# Autodesk Inventor assembly: Traction_Section
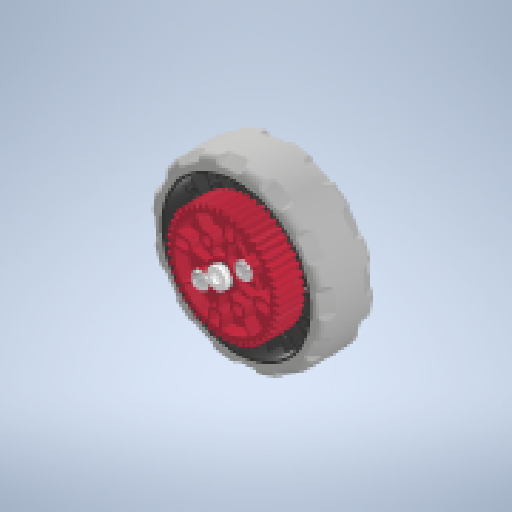
[picture p0: Inventor's stored thumbnail of the model, 512x512]
Saved by Autodesk Inventor 2025.2 (Build 292293000, 293)
## iProperties
Created: 2024-12-08
Part Number: Traction_Section
Document SubType Name: Assembly
Designer: Aditya Koduri
Author: Aditya Koduri
## Documents named in this file (13)
- C:\Users\joshi\Desktop\3388K CAD\Traction_Section.iam
- C:\Users\joshi\Desktop\3388K CAD\VEX Main\Structure\Hardware\Screw Steel - Hex\SScrew Hex Smooth 1.250.ipt
- C:\Users\joshi\Desktop\3388K CAD\VEX Main\Motion\Gears\HS Gear\HS 48T Gear, No Insert.iam
- C:\Users\joshi\Desktop\3388K CAD\VEX Main\Structure\Hardware\Nut Thin Nylock.ipt
- C:\Users\joshi\Desktop\3388K CAD\VEX Main\Motion\Wheels\Traction Wheel\3.25 Traction AS, No Insert.iam
- C:\Users\joshi\Desktop\3388K CAD\VEX Main\Motion\Insert Circle.ipt
- C:\Users\joshi\Desktop\3388K CAD\VEX Main\Motion\Spacers\Washer Teflon\TWasher .375 OD x .03125.ipt
- C:\Users\joshi\Desktop\3388K CAD\VEX Main\Motion\Spacers\Spacer Nylon .313 OD\NSpacer .313 OD x .250.ipt
- C:\Users\mzart\Downloads\VEX-CAD-Inventor-main\VEX-CAD-Inventor-main\Motion\Gears\HS Gear.iam
- C:\Users\mzart\Downloads\VEX-CAD-Inventor-main\VEX-CAD-Inventor-main\Motion\Spacers\Washer Teflon.ipt
- C:\Users\mzart\Downloads\VEX-CAD-Inventor-main\VEX-CAD-Inventor-main\Motion\Spacers\Spacer Nylon .313 OD.ipt
- C:\Users\mzart\Downloads\VEX-CAD-Inventor-main\VEX-CAD-Inventor-main\Motion\Wheels\Traction Wheel.iam
- C:\Users\mzart\Downloads\VEX-CAD-Inventor-main\VEX-CAD-Inventor-main\Structure\Hardware\Screw Steel - Hex.ipt
## Components (13 placed, 7 different names)
1. HS 48T Gear, No Insert:1 [sub-assembly] — Insert:14, Insert:15, Insert:16
2. Nut Thin Nylock:1 — Insert:19
3. Nut Thin Nylock:2 — Insert:18
4. Insert Circle:1
5. Insert Circle:2 — Insert:17
6. TWasher .375 OD x .03125:1
7. TWasher .375 OD x .03125:2
8. NSpacer .313 OD x .250:1
9. TWasher .375 OD x .03125:3
10. TWasher .375 OD x .03125:4
11. 3.25 Traction AS, No Insert:1 [sub-assembly] — Insert:14, Insert:17, Insert:18, Insert:19
12. SScrew Hex Smooth 1.250:1 — Insert:15
13. SScrew Hex Smooth 1.250:2 — Insert:16
## Relationships (12: Insert 12)
- [Insert]: HS 48T Gear, No Insert:1 ↔ Insert Circle:1
- [Insert]: Insert Circle:1 ↔ TWasher .375 OD x .03125:2
- [Insert]: TWasher .375 OD x .03125:1 ↔ TWasher .375 OD x .03125:2
- [Insert]: NSpacer .313 OD x .250:1 ↔ TWasher .375 OD x .03125:3
- [Insert]: Insert Circle:2 ↔ NSpacer .313 OD x .250:1
- [Insert]: TWasher .375 OD x .03125:3 ↔ TWasher .375 OD x .03125:4
- Insert:14: HS 48T Gear, No Insert:1 ↔ 3.25 Traction AS, No Insert:1
- Insert:15: HS 48T Gear, No Insert:1 ↔ SScrew Hex Smooth 1.250:1
- Insert:16: HS 48T Gear, No Insert:1 ↔ SScrew Hex Smooth 1.250:2
- Insert:17: Insert Circle:2 ↔ 3.25 Traction AS, No Insert:1
- Insert:18: Nut Thin Nylock:2 ↔ 3.25 Traction AS, No Insert:1
- Insert:19: Nut Thin Nylock:1 ↔ 3.25 Traction AS, No Insert:1
